# Autodesk Inventor assembly: ASY ДМФ 040 кольцо под шпильки КОРМА
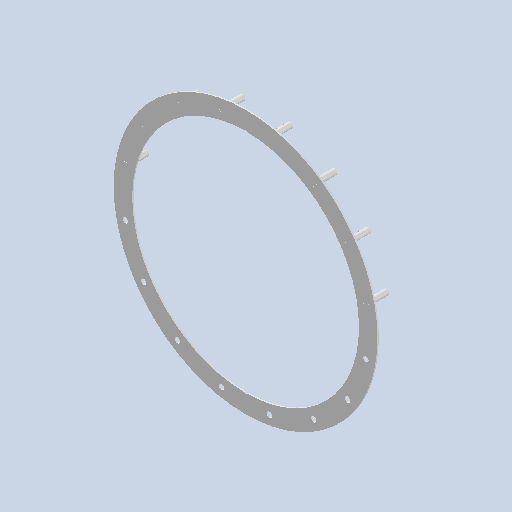
[picture p0: Inventor's stored thumbnail of the model, 512x512]
Saved by Autodesk Inventor 2025 (Build 290162010, 162A)
## iProperties
Created: 2024-05-08
Part Number: ASY ДМФ 040 кольцо под шпильки КОРМА
Document SubType Name: Assembly
Designer: pokla
Stock Number: ДМФ 040 кольцо под шпильки КОРМА
Author: pokla
## Documents named in this file (4)
- C:\Users\pokla\Documents\Inventor\ДФО\ДМФ\DMF-Disk-Micro-Filter\DMF old version\ASY ДМФ 040 кольцо под шпильки КОРМА.iam
- C:\Users\pokla\Documents\Inventor\ДФО\ДМФ\DMF-Disk-Micro-Filter\DMF old version\ДМФ 041 кольцо под шпильки КОРМА.ipt
- C:\Users\pokla\Documents\Inventor\ДФО\ДМФ\DMF-Disk-Micro-Filter\DMF old version\ДМФ 000 размеры.ipt
- C:\Users\pokla\Documents\Inventor\ДФО\ДМФ\DMF-Disk-Micro-Filter\DMF old version\ДМФ 043 шпилька 2.ipt
## Components (9 placed, 2 different names)
1. ДМФ 041 кольцо под шпильки КОРМА.ipt:1 — Rigid:2
2. ДМФ 043 шпилька 2.ipt:1 — Rigid:2
3. ДМФ 043 шпилька 2.ipt:2
4. ДМФ 043 шпилька 2.ipt:3
5. ДМФ 043 шпилька 2.ipt:4
6. ДМФ 043 шпилька 2.ipt:5
7. ДМФ 043 шпилька 2.ipt:6
8. ДМФ 043 шпилька 2.ipt:7
9. ДМФ 043 шпилька 2.ipt:8
## Component patterns: (8 elements, first: ДМФ 043 шпилька 2.ipt:1)
## Relationships (1: WeldJoint 1)
- Rigid:2 [WeldJoint]: ДМФ 041 кольцо под шпильки КОРМА.ipt:1 ↔ ДМФ 043 шпилька 2.ipt:1
